# Autodesk Inventor assembly: nc_nhk11
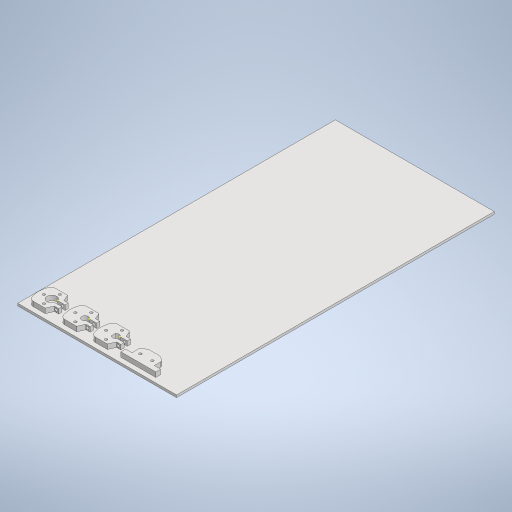
[picture p0: Inventor's stored thumbnail of the model, 512x512]
Saved by Autodesk Inventor 2023 (Build 270158000, 158)
## iProperties
Created: 2022-04-22
Part Number: nc_nhk11
Document SubType Name: Assembly
Designer: yuta
Author: yuta
## Documents named in this file (6)
- C:\Users\yuta\Documents\NHK\nc_nhk11.iam
- C:\Users\yuta\Documents\NHK\NC.port.ipt
- C:\Users\yuta\Documents\NHK\射出_腕固定.ipt
- C:\Users\yuta\Documents\NHK\射出_腕固定2.ipt
- C:\Users\yuta\Documents\NHK\射出_腕固定3.ipt
- C:\Users\yuta\Documents\NHK\射出_ベルト固定.ipt
## Components (5 placed, 5 different names)
1. NC.port:1 — メイト:1, フラッシュ:1, メイト:2, メイト:3, フラッシュ:2, メイト:5, フラッシュ:3, メイト:7, フラッシュ:4
2. 射出_腕固定:1 — メイト:1, フラッシュ:1, メイト:2, メイト:4
3. 射出_腕固定2:2 — メイト:3, フラッシュ:2, メイト:4, メイト:6
4. 射出_腕固定3:1 — メイト:5, フラッシュ:3, メイト:6, メイト:8
5. 射出_ベルト固定:1 — メイト:7, フラッシュ:4, メイト:8
## Relationships (12: Mate 8, Flush 4)
- メイト:1 [Mate]: NC.port:1 ↔ 射出_腕固定:1
- フラッシュ:1 [Flush] (6 mm): NC.port:1 ↔ 射出_腕固定:1
- メイト:2 [Mate] (-35 mm): NC.port:1 ↔ 射出_腕固定:1
- メイト:3 [Mate]: NC.port:1 ↔ 射出_腕固定2:2
- フラッシュ:2 [Flush] (6 mm): NC.port:1 ↔ 射出_腕固定2:2
- メイト:4 [Mate] (37 mm): 射出_腕固定:1 ↔ 射出_腕固定2:2
- メイト:5 [Mate]: NC.port:1 ↔ 射出_腕固定3:1
- フラッシュ:3 [Flush] (6 mm): NC.port:1 ↔ 射出_腕固定3:1
- メイト:6 [Mate] (36 mm): 射出_腕固定2:2 ↔ 射出_腕固定3:1
- メイト:7 [Mate]: NC.port:1 ↔ 射出_ベルト固定:1
- フラッシュ:4 [Flush] (6 mm): NC.port:1 ↔ 射出_ベルト固定:1
- メイト:8 [Mate] (8 mm): 射出_腕固定3:1 ↔ 射出_ベルト固定:1
